# Autodesk Inventor assembly: Moving Carousel Assembly
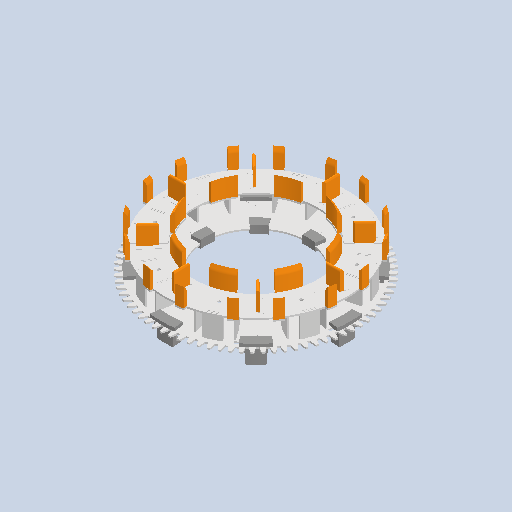
[picture p0: Inventor's stored thumbnail of the model, 512x512]
Saved by Autodesk Inventor 2023 (Build 270158000, 158)
## iProperties
Created: 2023-02-14
Part Number: Moving Carousel Assembly
Document SubType Name: Assembly
Designer: cheng
Mass: 4744.76 g
Surface Area: 15752.6 cm^2
Volume: 3946.5 cm^3
Density: 1.20227 g/cm^3
Author: cheng
## Documents named in this file (2)
- C:\Users\mihal\Desktop\4th Year Project\Final Assembly\Moving Carousel\Moving Carousel Assembly.iam
- C:\Users\mihal\Desktop\4th Year Project\Final Assembly\Moving Carousel\Moving Carousel Section Assembly.iam
## Components (8 placed, 1 different names)
1. Moving Carousel Section Assembly:1 [sub-assembly] — Mate:3, Flush:2, Mate:4, Mate:5, Flush:3, Mate:6, Mate:15
2. Moving Carousel Section Assembly:2 [sub-assembly] — Mate:1, Flush:1, Mate:2
3. Moving Carousel Section Assembly:3 [sub-assembly] — Mate:7, Flush:4, Mate:8, Mate:9, Flush:5, Mate:10
4. Moving Carousel Section Assembly:4 [sub-assembly] — Mate:5, Flush:3, Mate:6, Mate:7, Flush:4, Mate:8
5. Moving Carousel Section Assembly:5 [sub-assembly] — Mate:11, Flush:6, Mate:12, Mate:13, Flush:7, Mate:14
6. Moving Carousel Section Assembly:6 [sub-assembly] — Mate:13, Flush:7, Mate:14, Mate:16
7. Moving Carousel Section Assembly:7 [sub-assembly] — Mate:9, Flush:5, Mate:10, Mate:11, Flush:6, Mate:12
8. Moving Carousel Section Assembly:8 [sub-assembly] — Mate:1, Flush:1, Mate:2, Mate:3, Flush:2, Mate:4
## Relationships (23: Mate 16, Flush 7)
- Mate:1: Moving Carousel Section Assembly:2 ↔ Moving Carousel Section Assembly:8
- Flush:1: Moving Carousel Section Assembly:2 ↔ Moving Carousel Section Assembly:8
- Mate:2: Moving Carousel Section Assembly:2 ↔ Moving Carousel Section Assembly:8
- Mate:3: Moving Carousel Section Assembly:1 ↔ Moving Carousel Section Assembly:8
- Flush:2: Moving Carousel Section Assembly:1 ↔ Moving Carousel Section Assembly:8
- Mate:4: Moving Carousel Section Assembly:1 ↔ Moving Carousel Section Assembly:8
- Mate:5: Moving Carousel Section Assembly:1 ↔ Moving Carousel Section Assembly:4
- Flush:3: Moving Carousel Section Assembly:1 ↔ Moving Carousel Section Assembly:4
- Mate:6: Moving Carousel Section Assembly:1 ↔ Moving Carousel Section Assembly:4
- Mate:7: Moving Carousel Section Assembly:3 ↔ Moving Carousel Section Assembly:4
- Flush:4: Moving Carousel Section Assembly:3 ↔ Moving Carousel Section Assembly:4
- Mate:8: Moving Carousel Section Assembly:3 ↔ Moving Carousel Section Assembly:4
- Mate:9: Moving Carousel Section Assembly:3 ↔ Moving Carousel Section Assembly:7
- Flush:5: Moving Carousel Section Assembly:3 ↔ Moving Carousel Section Assembly:7
- Mate:10: Moving Carousel Section Assembly:3 ↔ Moving Carousel Section Assembly:7
- Mate:11: Moving Carousel Section Assembly:5 ↔ Moving Carousel Section Assembly:7
- Flush:6: Moving Carousel Section Assembly:5 ↔ Moving Carousel Section Assembly:7
- Mate:12: Moving Carousel Section Assembly:5 ↔ Moving Carousel Section Assembly:7
- Mate:13: Moving Carousel Section Assembly:5 ↔ Moving Carousel Section Assembly:6
- Flush:7: Moving Carousel Section Assembly:5 ↔ Moving Carousel Section Assembly:6
- Mate:14: Moving Carousel Section Assembly:5 ↔ Moving Carousel Section Assembly:6
- Mate:15: Moving Carousel Section Assembly:1
- Mate:16: Moving Carousel Section Assembly:6
